# Autodesk Inventor assembly: Antrieb und Differential
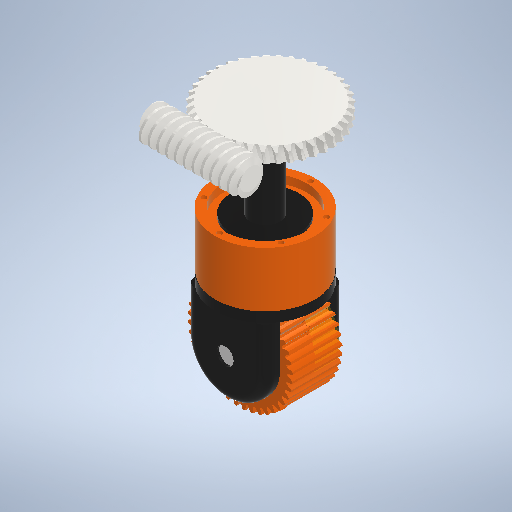
[picture p0: Inventor's stored thumbnail of the model, 512x512]
Saved by Autodesk Inventor 2025 (Build 290162010, 162A)
## iProperties
Created: 2024-11-13
Part Number: Antrieb und Differential
Document SubType Name: Assembly
Designer: jensb
Author: jensb
## Documents named in this file (11)
- C:\Users\jensb\Desktop\Projektarbeit\Bauteile\Antrieb und Differential.iam
- C:\Users\jensb\Desktop\Projektarbeit\Bauteile\CNS 397 - 3 x 6A.ipt
- C:\Users\jensb\Desktop\Projektarbeit\Bauteile\DIN 625 T1 - 6203 - 17 x 40 x 12.ipt
- C:\Users\jensb\Desktop\Projektarbeit\Bauteile\Rundstab 17 x 75.ipt
- C:\Users\jensb\Desktop\Projektarbeit\Bauteile\Stirnzahnrad11.ipt
- C:\Users\jensb\Desktop\Projektarbeit\Bauteile\Stirnzahnrad21.ipt
- C:\Users\jensb\Desktop\Projektarbeit\Bauteile\DIN 625 T1 - 625 - 5 x 16 x 5.ipt
- C:\Users\jensb\Desktop\Projektarbeit\Bauteile\Haltevorrichtung1.ipt
- C:\Users\jensb\Desktop\Projektarbeit\Bauteile\Innerer Differential Wurm Getriebe.ipt
- C:\Users\jensb\Desktop\Projektarbeit\Bauteile\Haltevorrichtung2.ipt
- C:\Users\jensb\Desktop\Projektarbeit\Bauteile\Antrieb und Differential\Konstruktions-Assistent\Schneckenräder1.iam
## Components (15 placed, 10 different names)
1. Haltevorrichtung1:1 — Passend:27, Passend:28, Passend:29, Passend:30, Passend:31, Passend:32, Passend:35
2. Haltevorrichtung2:1 — Passend:33, Passend:34, Passend:35
3. Innerer Differential Wurm Getriebe:1 — Passend:31, Passend:32, Drehung:2
4. Schneckenräder:1 [sub-assembly]
5. Rundstab 17 x 75:1 — Passend:5, Fluchtend:1, Passend:27, Passend:33
6. CNS 397 A 3 x 6:1 — Winkel:3, Winkel:4, Winkel:5, Passend:1, Passend:11, Passend:13, Winkel:8, Winkel:9, Winkel:10, Winkel:11
7. CNS 397 A 3 x 6:2 — Winkel:5, Passend:3, Passend:14, Winkel:10
8. CNS 397 A 3 x 6:3 — Winkel:4, Passend:4, Passend:15, Winkel:9
9. CNS 397 A 3 x 6:4 — Winkel:3, Passend:2, Passend:16, Winkel:8
10. DIN 625 - T1 6203 - 17 x 40 x 12:2 — Passend:8, Passend:9, Winkel:12
11. DIN 625 - T1 6203 - 17 x 40 x 12:1 — Passend:5, Fluchtend:1, Passend:6, Passend:7, Winkel:12, Passend:18
12. Stirnzahnrad1:2 — Passend:8, Passend:9, Passend:10, Passend:11, Passend:12
13. Stirnzahnrad1:1 — Passend:1, Passend:2, Passend:3, Passend:4, Passend:6, Passend:7, Passend:10, Passend:12, Passend:13, Passend:14, Passend:15, Passend:16, Winkel:11, Passend:18, Passend:19, Tangential:1, Passend:24, Passend:25, Passend:26, Drehung:1, Passend:28
14. DIN 625 - T1 625 - 5 x 16 x 5:1 — Passend:23, Fluchtend:2, Passend:29, Winkel:13, Passend:34
15. Stirnzahnrad2:1 — Passend:19, Passend:23, Fluchtend:2, Tangential:1, Drehung:1, Winkel:13, Drehung:2
## Relationships (45: Mate 31, Angle 9, Flush 2, RelateRotation 2, Tangent 1)
- Winkel:3 [Angle] (0 deg): CNS 397 A 3 x 6:1 ↔ CNS 397 A 3 x 6:4
- Winkel:4 [Angle] (0 deg): CNS 397 A 3 x 6:1 ↔ CNS 397 A 3 x 6:3
- Winkel:5 [Angle] (0 deg): CNS 397 A 3 x 6:1 ↔ CNS 397 A 3 x 6:2
- Passend:1 [Mate]: CNS 397 A 3 x 6:1 ↔ Stirnzahnrad1:1
- Passend:2 [Mate]: CNS 397 A 3 x 6:4 ↔ Stirnzahnrad1:1
- Passend:3 [Mate]: CNS 397 A 3 x 6:2 ↔ Stirnzahnrad1:1
- Passend:4 [Mate]: CNS 397 A 3 x 6:3 ↔ Stirnzahnrad1:1
- Passend:5 [Mate]: Rundstab 17 x 75:1 ↔ DIN 625 - T1 6203 - 17 x 40 x 12:1
- Fluchtend:1 [Flush] (-12.5 mm): Rundstab 17 x 75:1 ↔ DIN 625 - T1 6203 - 17 x 40 x 12:1
- Passend:6 [Mate]: DIN 625 - T1 6203 - 17 x 40 x 12:1 ↔ Stirnzahnrad1:1
- Passend:7 [Mate]: DIN 625 - T1 6203 - 17 x 40 x 12:1 ↔ Stirnzahnrad1:1
- Passend:8 [Mate]: DIN 625 - T1 6203 - 17 x 40 x 12:2 ↔ Stirnzahnrad1:2
- Passend:9 [Mate]: DIN 625 - T1 6203 - 17 x 40 x 12:2 ↔ Stirnzahnrad1:2
- Passend:10 [Mate]: Stirnzahnrad1:2 ↔ Stirnzahnrad1:1
- Passend:11 [Mate]: CNS 397 A 3 x 6:1 ↔ Stirnzahnrad1:2
- Passend:12 [Mate]: Stirnzahnrad1:2 ↔ Stirnzahnrad1:1
- Passend:13 [Mate]: CNS 397 A 3 x 6:1 ↔ Stirnzahnrad1:1
- Passend:14 [Mate]: CNS 397 A 3 x 6:2 ↔ Stirnzahnrad1:1
- Passend:15 [Mate]: CNS 397 A 3 x 6:3 ↔ Stirnzahnrad1:1
- Passend:16 [Mate]: CNS 397 A 3 x 6:4 ↔ Stirnzahnrad1:1
- Winkel:8 [Angle] (0 deg): CNS 397 A 3 x 6:1 ↔ CNS 397 A 3 x 6:4
- Winkel:9 [Angle] (0 deg): CNS 397 A 3 x 6:1 ↔ CNS 397 A 3 x 6:3
- Winkel:10 [Angle] (0 deg): CNS 397 A 3 x 6:1 ↔ CNS 397 A 3 x 6:2
- Winkel:11 [Angle] (0 deg): CNS 397 A 3 x 6:1 ↔ Stirnzahnrad1:1
- Winkel:12 [Angle] (0 deg): DIN 625 - T1 6203 - 17 x 40 x 12:2 ↔ DIN 625 - T1 6203 - 17 x 40 x 12:1
- Passend:18 [Mate]: DIN 625 - T1 6203 - 17 x 40 x 12:1 ↔ Stirnzahnrad1:1
- Passend:19 [Mate] (2.5 mm): Stirnzahnrad1:1 ↔ Stirnzahnrad2:1
- Passend:23 [Mate]: DIN 625 - T1 625 - 5 x 16 x 5:1 ↔ Stirnzahnrad2:1
- Fluchtend:2 [Flush]: DIN 625 - T1 625 - 5 x 16 x 5:1 ↔ Stirnzahnrad2:1
- Tangential:1: Stirnzahnrad1:1 ↔ Stirnzahnrad2:1
- Passend:24 [Mate]: Stirnzahnrad1:1
- Passend:25 [Mate]: Stirnzahnrad1:1
- Passend:26 [Mate]: Stirnzahnrad1:1
- Drehung:1 [RelateRotation] (2 ul): Stirnzahnrad1:1 ↔ Stirnzahnrad2:1
- Passend:27 [Mate]: Haltevorrichtung1:1 ↔ Rundstab 17 x 75:1
- Passend:28 [Mate]: Haltevorrichtung1:1 ↔ Stirnzahnrad1:1
- Passend:29 [Mate]: Haltevorrichtung1:1 ↔ DIN 625 - T1 625 - 5 x 16 x 5:1
- Passend:30 [Mate]: Haltevorrichtung1:1
- Winkel:13 [Angle] (0 deg): DIN 625 - T1 625 - 5 x 16 x 5:1 ↔ Stirnzahnrad2:1
- Passend:31 [Mate]: Haltevorrichtung1:1 ↔ Innerer Differential Wurm Getriebe:1
- Passend:32 [Mate]: Haltevorrichtung1:1 ↔ Innerer Differential Wurm Getriebe:1
- Drehung:2 [RelateRotation] (20 ul): Innerer Differential Wurm Getriebe:1 ↔ Stirnzahnrad2:1
- Passend:33 [Mate]: Haltevorrichtung2:1 ↔ Rundstab 17 x 75:1
- Passend:34 [Mate]: Haltevorrichtung2:1 ↔ DIN 625 - T1 625 - 5 x 16 x 5:1
- Passend:35 [Mate]: Haltevorrichtung1:1 ↔ Haltevorrichtung2:1
